# Autodesk Inventor assembly: mecanum_adaptive_trajectory
(part 2 of 2)
- 挿入:304 [Insert]: mecanum_encoder_plateD:1 ↔ mecanum_encoder_shaftD:1
- 挿入:305 [Insert]: mecanum_encoder_plateD:1 ↔ mecanum_encoder_shaftD:2
- 挿入:306 [Insert]: mecanum_encoder_plateD:1 ↔ mecanum_encoder_shaftD:3
- 挿入:307 [Insert]: mecanum_encoder_shaftD:1 ↔ mecanum_encoder_plateC:3
- 挿入:308 [Insert]: mecanum_encoder_shaftD:2 ↔ mecanum_encoder_plateC:3
- 挿入:309 [Insert]: mecanum_encoder_shaftD:3 ↔ mecanum_encoder_plateC:3
- メイト:77 [Mate]: mecanum_encoder_shaftA:1 ↔ mecanum_encoder_coupling:1
- メイト:78 [Mate] (4 mm): mecanum_encoder_plateC:1 ↔ mecanum_encoder_coupling:1
- メイト:79 [Mate]: Astuto_enc_wheel:2 ↔ mecanum_encoder_coupling:2
- メイト:80 [Mate] (5 mm): mecanum_encoder_plateC:2 ↔ mecanum_encoder_coupling:2
- メイト:81 [Mate]: Astuto_enc_wheel:2 ↔ mecanum_encoder_shaftE:1
- フラッシュ:6 [Flush] (10.609 mm): Astuto_enc_part3:2 ↔ Astuto_enc_part2:4
- フラッシュ:7 [Flush] (5 mm): mecanum_encoder_plateD:1 ↔ mecanum_encoder_shaftE:1
- [Insert]: E6A2-CW3C:3 ↔ mecanum_encoder_plateC:4
- [Insert]: E6A2-CW3C:3 ↔ mecanum_encoder_plateC:4
- [Mate]: Astuto_enc_part3:3 ↔ Astuto_enc_part2:7
- [Mate]: Astuto_enc_part3:4 ↔ Astuto_enc_part2:6
- [Mate] (0.2 mm): Astuto_enc_part3:3 ↔ Astuto_enc_part2:7
- [Mate] (0.2 mm): Astuto_enc_part3:4 ↔ Astuto_enc_part2:6
- [Insert]: Astuto_enc_part2:6 ↔ mecanum_encoder_plateD:2
- [Insert]: Astuto_enc_part2:7 ↔ mecanum_encoder_plateD:2
- [Insert]: Astuto_enc_part2:7 ↔ mecanum_encoder_plateD:2
- [Insert]: Astuto_enc_part2:6 ↔ mecanum_encoder_plateD:2
- [Mate]: Astuto_enc_wheel:3 ↔ mecanum_encoder_plateD:2
- [Insert]: mecanum_encoder_plateD:2 ↔ mecanum_encoder_shaftD:4
- [Insert]: mecanum_encoder_plateD:2 ↔ mecanum_encoder_shaftD:5
- [Insert]: mecanum_encoder_plateD:2 ↔ mecanum_encoder_shaftD:6
- [Insert]: mecanum_encoder_shaftD:4 ↔ mecanum_encoder_plateC:5
- [Insert]: mecanum_encoder_shaftD:5 ↔ mecanum_encoder_plateC:5
- [Insert]: mecanum_encoder_shaftD:6 ↔ mecanum_encoder_plateC:5
- [Mate]: Astuto_enc_wheel:3 ↔ mecanum_encoder_coupling:3
- [Mate] (5 mm): mecanum_encoder_plateC:4 ↔ mecanum_encoder_coupling:3
- [Mate]: Astuto_enc_wheel:3 ↔ mecanum_encoder_shaftE:2
- [Flush] (10.609 mm): Astuto_enc_part3:4 ↔ Astuto_enc_part2:6
- [Flush] (5 mm): mecanum_encoder_plateD:2 ↔ mecanum_encoder_shaftE:2
- 挿入:331 [Insert]: mecanum_flameD:1 ↔ Astuto_enc_part3:3
- 挿入:332 [Insert]: mecanum_flameD:2 ↔ Astuto_enc_part3:3
- 挿入:333 [Insert]: mecanum_flameD:2 ↔ Astuto_enc_part3:4
- 挿入:334 [Insert]: mecanum_flameD:1 ↔ Astuto_enc_part3:4
- メイト:91 [Mate] (5 mm): Astuto_enc_wheel:1 ↔ mecanum_encoder_plateA:1
- [Mate]: Astuto_enc_wheel:4 ↔ mecanum_encoder_shaftA:2
- [Mate]: mecanum_encoder_shaftA:2 ↔ mecanum_encoder_plateB:2
- [Mate]: Astuto_enc_part1:4 ↔ Astuto_enc_part2:8
- [Mate] (0.2 mm): Astuto_enc_part1:4 ↔ Astuto_enc_part2:8
- [Insert]: mecanum_encoder_plateB:2 ↔ Astuto_enc_part2:8
- [Insert]: mecanum_encoder_plateB:2 ↔ Astuto_enc_part2:8
- [Mate]: Astuto_enc_part1:5 ↔ Astuto_enc_part2:9
- [Insert]: mecanum_encoder_plateB:2 ↔ Astuto_enc_part2:9
- [Insert]: mecanum_encoder_plateB:2 ↔ Astuto_enc_part2:9
- [Mate] (0.2 mm): Astuto_enc_part1:5 ↔ Astuto_enc_part2:9
- [Flush] (17.307 mm): Astuto_enc_part1:4 ↔ Astuto_enc_part2:8
- [Mate]: mecanum_encoder_shaftA:2 ↔ mecanum_encoder_plateA:2
- [Insert]: mecanum_encoder_plateB:2 ↔ mecanum_encoder_shaftB:3
- [Insert]: mecanum_encoder_plateA:2 ↔ mecanum_encoder_shaftB:3
- [Insert]: mecanum_encoder_plateA:2 ↔ mecanum_encoder_shaftB:4
- [Insert]: E6A2-CW3C:4 ↔ mecanum_encoder_plateC:6
- [Insert]: E6A2-CW3C:4 ↔ mecanum_encoder_plateC:6
- [Mate]: mecanum_encoder_shaftA:2 ↔ E6A2-CW3C:4
- [Flush] (6 mm): mecanum_encoder_shaftA:2 ↔ mecanum_encoder_plateA:2
- [Insert]: mecanum_encoder_plateC:6 ↔ mecanum_encoder_shaftC:10
- [Insert]: mecanum_encoder_plateC:6 ↔ mecanum_encoder_shaftC:12
- [Insert]: mecanum_encoder_plateC:6 ↔ mecanum_encoder_shaftC:11
- [Mate]: mecanum_encoder_plateB:2 ↔ mecanum_encoder_shaftC:10
- [Insert]: mecanum_encoder_plateB:2 ↔ mecanum_encoder_shaftC:12
- [Insert]: mecanum_encoder_plateB:2 ↔ mecanum_encoder_shaftC:10
- [Insert]: mecanum_encoder_plateB:2 ↔ mecanum_encoder_shaftC:11
- [Mate]: mecanum_encoder_shaftA:2 ↔ mecanum_encoder_coupling:4
- [Mate] (4 mm): mecanum_encoder_plateC:6 ↔ mecanum_encoder_coupling:4
- [Mate] (5 mm): Astuto_enc_wheel:4 ↔ mecanum_encoder_plateA:2
- 挿入:350 [Insert]: mecanum_flameB_MIR:1 ↔ Astuto_enc_part1:4
- 挿入:351 [Insert]: mecanum_flameB_MIR:4 ↔ Astuto_enc_part1:4
- 挿入:352 [Insert]: mecanum_flameB_MIR:4 ↔ Astuto_enc_part1:5
- 挿入:353 [Insert]: mecanum_flameB_MIR:1 ↔ Astuto_enc_part1:5
- メイト:105 [Mate] (6.15 mm): Astuto_enc_wheel:2 ↔ mecanum_encoder_plateD:1
- メイト:106 [Mate] (6.15 mm): Astuto_enc_wheel:3 ↔ mecanum_encoder_plateD:2
- 挿入:354 [Insert]: mecanum_encoder_plateC:5 ↔ mecanum_encoder_shaftF:1
- 挿入:355 [Insert]: mecanum_encoder_plateC:4 ↔ mecanum_encoder_shaftF:1
- 挿入:356 [Insert]: mecanum_encoder_plateC:4 ↔ mecanum_encoder_shaftF:2
- 挿入:357 [Insert]: mecanum_encoder_plateC:4 ↔ mecanum_encoder_shaftF:3
- 挿入:358 [Insert]: mecanum_encoder_plateC:5 ↔ mecanum_encoder_shaftF:2
- 挿入:359 [Insert]: mecanum_encoder_plateC:5 ↔ mecanum_encoder_shaftF:3
- 挿入:360 [Insert]: mecanum_encoder_plateC:3 ↔ mecanum_encoder_shaftF:4
- 挿入:361 [Insert]: mecanum_encoder_plateC:2 ↔ mecanum_encoder_shaftF:4
- 挿入:362 [Insert]: mecanum_encoder_plateC:2 ↔ mecanum_encoder_shaftF:5
- 挿入:363 [Insert]: mecanum_encoder_plateC:2 ↔ mecanum_encoder_shaftF:6
- 挿入:364 [Insert]: mecanum_encoder_plateC:3 ↔ mecanum_encoder_shaftF:5
- 挿入:365 [Insert]: mecanum_encoder_plateC:3 ↔ mecanum_encoder_shaftF:6
- 挿入:372 [Insert]: mecanum_flameB_MIR:2 ↔ mecanum_flameF:1
- 挿入:373 [Insert]: mecanum_flameB_MIR:3 ↔ mecanum_flameF:1
- 挿入:374 [Insert]: mecanum_flameB_MIR:2 ↔ mecanum_flameF:2
- 挿入:375 [Insert]: mecanum_flameB_MIR:3 ↔ mecanum_flameF:2
- 挿入:377 [Insert]: mecanum_flameF:1 ↔ mecanum_LRF_flameA:1
- 挿入:379 [Insert]: mecanum_flameF:2 ↔ mecanum_LRF_flameA:2
- 挿入:384 [Insert]: LRF:1 ↔ mecanum_LRF_plate:1
- 挿入:385 [Insert]: LRF:1 ↔ mecanum_LRF_plate:1
- 挿入:386 [Insert]: LRF:1 ↔ mecanum_LRF_plate:1
- 挿入:387 [Insert]: LRF:1 ↔ mecanum_LRF_plate:1
- 挿入:388 [Insert]: mecanum_LRF_flameA:1 ↔ mecanum_LRF_plate:1
- 挿入:389 [Insert]: mecanum_LRF_flameA:1 ↔ mecanum_LRF_plate:1
- 挿入:390 [Insert]: mecanum_LRF_flameA:2 ↔ mecanum_LRF_plate:1
- 挿入:391 [Insert]: mecanum_LRF_flameA:2 ↔ mecanum_LRF_plate:1
- 挿入:392 [Insert]: mecanum_LRF_flameA:1 ↔ mecanum_gusset_plateA:1
- 挿入:393 [Insert]: mecanum_LRF_flameA:1 ↔ mecanum_gusset_plateA:1
- 挿入:394 [Insert]: mecanum_flameF:1 ↔ mecanum_LRF_flameB:1
- 挿入:395 [Insert]: mecanum_gusset_plateA:1 ↔ mecanum_LRF_flameB:1
- 挿入:396 [Insert]: mecanum_gusset_plateA:1 ↔ mecanum_LRF_flameB:1
- 挿入:397 [Insert]: mecanum_LRF_flameA:2 ↔ mecanum_gusset_plateA:2
- 挿入:398 [Insert]: mecanum_LRF_flameA:2 ↔ mecanum_gusset_plateA:2
- 挿入:399 [Insert]: mecanum_gusset_plateA:2 ↔ mecanum_LRF_flameB:2
- 挿入:400 [Insert]: mecanum_gusset_plateA:2 ↔ mecanum_LRF_flameB:2
- 挿入:401 [Insert]: mecanum_flameF:2 ↔ mecanum_LRF_flameB:2
- [Insert]: mecanum_flameF:3 ↔ mecanum_LRF_flameA:3
- [Insert]: mecanum_flameF:4 ↔ mecanum_LRF_flameA:4
- [Insert]: LRF:3 ↔ mecanum_LRF_plate:2
- [Insert]: LRF:3 ↔ mecanum_LRF_plate:2
- [Insert]: LRF:3 ↔ mecanum_LRF_plate:2
- [Insert]: LRF:3 ↔ mecanum_LRF_plate:2
- [Insert]: mecanum_LRF_flameA:3 ↔ mecanum_LRF_plate:2
- [Insert]: mecanum_LRF_flameA:3 ↔ mecanum_LRF_plate:2
- [Insert]: mecanum_LRF_flameA:4 ↔ mecanum_LRF_plate:2
- [Insert]: mecanum_LRF_flameA:4 ↔ mecanum_LRF_plate:2
- [Insert]: mecanum_LRF_flameA:3 ↔ mecanum_gusset_plateA:3
- [Insert]: mecanum_LRF_flameA:3 ↔ mecanum_gusset_plateA:3
- [Insert]: mecanum_flameF:3 ↔ mecanum_LRF_flameB:3
- [Insert]: mecanum_gusset_plateA:3 ↔ mecanum_LRF_flameB:3
- [Insert]: mecanum_gusset_plateA:3 ↔ mecanum_LRF_flameB:3
- [Insert]: mecanum_LRF_flameA:4 ↔ mecanum_gusset_plateA:4
- [Insert]: mecanum_LRF_flameA:4 ↔ mecanum_gusset_plateA:4
- [Insert]: mecanum_gusset_plateA:4 ↔ mecanum_LRF_flameB:4
- [Insert]: mecanum_gusset_plateA:4 ↔ mecanum_LRF_flameB:4
- [Insert]: mecanum_flameF:4 ↔ mecanum_LRF_flameB:4
- 挿入:422 [Insert]: mecanum_flameB:2 ↔ mecanum_flameF:3
- 挿入:423 [Insert]: mecanum_flameB:3 ↔ mecanum_flameF:3
- 挿入:424 [Insert]: mecanum_flameB:2 ↔ mecanum_flameF:4
- 挿入:425 [Insert]: mecanum_flameB:3 ↔ mecanum_flameF:4
- 挿入:426 [Insert]: mecanum_flameB_MIR:2 ↔ mecanum_LRF_flameA:2
- 挿入:427 [Insert]: mecanum_flameB_MIR:2 ↔ mecanum_LRF_flameA:1
- 挿入:428 [Insert]: mecanum_flameB:2 ↔ mecanum_LRF_flameA:3
- 挿入:429 [Insert]: mecanum_flameB:2 ↔ mecanum_LRF_flameA:4
- メイト:107 [Mate]: mecanum_angleA:2 ↔ mecanum_kusaA:2
- フラッシュ:13 [Flush]: mecanum_angleA:2 ↔ mecanum_kusaA:2
- フラッシュ:14 [Flush]: mecanum_angleA:2 ↔ mecanum_kusaA:2
- フラッシュ:15 [Flush]: mecanum_angleA:1 ↔ mecanum_kusaA:1
- フラッシュ:16 [Flush]: mecanum_angleA:1 ↔ mecanum_kusaA:1
- メイト:108 [Mate]: mecanum_angleA:1 ↔ mecanum_kusaA:1
- メイト:109 [Mate]: mecanum_angleB:2 ↔ mecanum_kusaB:1
- フラッシュ:17 [Flush]: mecanum_angleB:2 ↔ mecanum_kusaB:1
- フラッシュ:18 [Flush]: mecanum_angleB:2 ↔ mecanum_kusaB:1
- フラッシュ:19 [Flush]: mecanum_angleB:1 ↔ mecanum_kusaB:2
- フラッシュ:20 [Flush]: mecanum_angleB:1 ↔ mecanum_kusaB:2
- メイト:110 [Mate]: mecanum_angleB:1 ↔ mecanum_kusaB:2
- 挿入:430 [Insert]: mecanum_flameB:2 ↔ mecanum_flameG:1
- 挿入:431 [Insert]: mecanum_flameE:1 ↔ mecanum_flameG:1
- 挿入:432 [Insert]: motor_plate:1 ↔ mecanum_flameG:1
- 挿入:433 [Insert]: motor_plate:1 ↔ mecanum_flameG:1
- 挿入:434 [Insert]: mecanum_flameB:1 ↔ mecanum_flameG:1
- 挿入:435 [Insert]: mecanum_flameE:5 ↔ mecanum_flameG:1
- 挿入:436 [Insert]: mecanum_flameE_MIR:5 ↔ mecanum_flameG:1
- 挿入:437 [Insert]: mecanum_flameB_MIR:1 ↔ mecanum_flameG:1
- 挿入:438 [Insert]: motor_plate_MIR1:1 ↔ mecanum_flameG:1
- 挿入:439 [Insert]: motor_plate_MIR1:1 ↔ mecanum_flameG:1
- 挿入:440 [Insert]: mecanum_flameB_MIR:2 ↔ mecanum_flameG:1
- 挿入:441 [Insert]: mecanum_flameE_MIR:1 ↔ mecanum_flameG:1
- 挿入:442 [Insert]: mecanum_flameE:1 ↔ mecanum_flameG:2
- 挿入:443 [Insert]: mecanum_flameB:3 ↔ mecanum_flameG:2
- 挿入:444 [Insert]: motor_plate:1 ↔ mecanum_flameG:2
- 挿入:445 [Insert]: motor_plate:1 ↔ mecanum_flameG:2
- 挿入:446 [Insert]: mecanum_flameB:4 ↔ mecanum_flameG:2
- 挿入:447 [Insert]: mecanum_flameB:3 ↔ mecanum_flameG:2
- 挿入:448 [Insert]: mecanum_flameE:1 ↔ mecanum_flameG:2
- 挿入:449 [Insert]: mecanum_flameE:5 ↔ mecanum_flameG:2
- 挿入:450 [Insert]: mecanum_flameB_MIR:4 ↔ mecanum_flameG:2
- 挿入:451 [Insert]: mecanum_flameE_MIR:5 ↔ mecanum_flameG:2
- 挿入:452 [Insert]: motor_plate_MIR1:1 ↔ mecanum_flameG:2
- 挿入:453 [Insert]: motor_plate_MIR1:1 ↔ mecanum_flameG:2
- 挿入:454 [Insert]: mecanum_flameB_MIR:3 ↔ mecanum_flameG:2
- 挿入:455 [Insert]: mecanum_flameE_MIR:1 ↔ mecanum_flameG:2
- 挿入:456 [Insert]: mecanum_flameE_MIR:3 ↔ mecanum_flameG:3
- 挿入:457 [Insert]: mecanum_flameB_MIR:3 ↔ mecanum_flameG:3
- 挿入:458 [Insert]: motor_plate_MIR_MIR:1 ↔ mecanum_flameG:3
- 挿入:459 [Insert]: mecanum_flameE_MIR:6 ↔ mecanum_flameG:3
- 挿入:460 [Insert]: mecanum_flameB:4 ↔ mecanum_flameG:3
- 挿入:461 [Insert]: mecanum_flameE:6 ↔ mecanum_flameG:3
- 挿入:462 [Insert]: motor_plate_MIR:1 ↔ mecanum_flameG:3
- 挿入:463 [Insert]: motor_plate_MIR:1 ↔ mecanum_flameG:3
- 挿入:464 [Insert]: mecanum_flameB:3 ↔ mecanum_flameG:3
- 挿入:465 [Insert]: mecanum_flameB:3 ↔ mecanum_flameE:3
- 挿入:466 [Insert]: mecanum_flameE_MIR:3 ↔ mecanum_flameG:4
- 挿入:467 [Insert]: mecanum_flameB_MIR:2 ↔ mecanum_flameG:4
- 挿入:468 [Insert]: motor_plate_MIR_MIR:1 ↔ mecanum_flameG:4
- 挿入:469 [Insert]: motor_plate_MIR_MIR:1 ↔ mecanum_flameG:4
- 挿入:470 [Insert]: mecanum_flameB_MIR:1 ↔ mecanum_flameG:4
- 挿入:471 [Insert]: mecanum_flameE_MIR:6 ↔ mecanum_flameG:4
- 挿入:472 [Insert]: mecanum_flameB:1 ↔ mecanum_flameG:4
- 挿入:473 [Insert]: mecanum_flameE:6 ↔ mecanum_flameG:4
- 挿入:474 [Insert]: motor_plate_MIR:1 ↔ mecanum_flameG:4
- 挿入:475 [Insert]: motor_plate_MIR:1 ↔ mecanum_flameG:4
- 挿入:476 [Insert]: mecanum_flameB:2 ↔ mecanum_flameG:4
- 挿入:477 [Insert]: mecanum_flameE:3 ↔ mecanum_flameG:4
- 挿入:478 [Insert]: mecanum_flameG:4 ↔ mecanum_flameH:1
- 挿入:479 [Insert]: mecanum_flameG:1 ↔ mecanum_flameH:1
- 挿入:480 [Insert]: mecanum_flameG:4 ↔ mecanum_flameH:2
- 挿入:481 [Insert]: mecanum_flameG:1 ↔ mecanum_flameH:2
- 挿入:482 [Insert]: mecanum_flameH:1 ↔ mecanum_suction_motor_plate:1
- 挿入:483 [Insert]: mecanum_suction_motor_plate:1 ↔ mecanum_flameH:2
- 挿入:484 [Insert]: mecanum_flameH:1 ↔ mecanum_suction_motor_plate:1
- 挿入:485 [Insert]: mecanum_suction_motor_plate:1 ↔ mecanum_flameH:2
- 挿入:486 [Insert]: fan_冶具-01:1 ↔ mecanum_suction_motor_plate:1
- 挿入:487 [Insert]: fan_冶具-01:1 ↔ mecanum_suction_motor_plate:1
- 挿入:488 [Insert]: fan_冶具-01:1 ↔ mecanum_suction_motor_plate:1
- 挿入:489 [Insert]: fan_冶具-01:1 ↔ mecanum_suction_motor_plate:1
- 挿入:490 [Insert]: fan_冶具-01:1 ↔ mecanum_suction_motor_plate:1
- 挿入:491 [Insert]: fan_冶具-01:2 ↔ mecanum_suction_motor_plate:1
- 挿入:492 [Insert]: fan_冶具-01:2 ↔ mecanum_suction_motor_plate:1
- 挿入:493 [Insert]: fan_冶具-01:2 ↔ mecanum_suction_motor_plate:1
- 挿入:494 [Insert]: fan_冶具-01:2 ↔ mecanum_suction_motor_plate:1
- メイト:111 [Mate]: 14-KEY-RZ-735:1 ↔ mecanum_shaft:1
- メイト:112 [Mate]: 14-KEY-RZ-736_MIR:1 ↔ mecanum_shaft_MIR:1
- メイト:113 [Mate]: 14-KEY-RZ-736_MIR1:1 ↔ mecanum_shaft_MIR1:1
- メイト:114 [Mate]: 14-KEY-RZ-736_MIR_MIR:1 ↔ mecanum_shaft_MIR_MIR:1
## Named parameters: d291_d278 = 0 mm, d292_d280 = 0 mm, d293_d281 = 0 mm, d294_d282 = 0 mm, d295_d283 = 0 mm, d296_d288 = 0 mm, d297_d289 = 0 mm, d298_d290 = 0 mm, d306_d278 = 0 mm, d307_d280 = 0 mm, d308_d281 = 0 mm, d309_d282 = 0 mm, d310_d283 = 0 mm, d311_d288 = 0 mm, d312_d289 = 0 mm, d313_d290 = 0 mm, d314_d278 = 0 mm, d315_d280 = 0 mm, d316_d281 = 0 mm, d317_d282 = 0 mm, d318_d283 = 0 mm, d319_d288 = 0 mm, d320_d289 = 0 mm, d321_d290 = 0 mm, d343_d339 = 0 mm, d382_d368 = 0 mm, d383_d369 = 0 mm, d425_d423 = 10 mm, d426_d424 = 5 mm, d427_d402 = 0 mm, d428_d403 = 0 mm, d429_d404 = 0 mm, d430_d405 = 0 mm, d431_d406 = 0 mm, d432_d407 = 0 mm, d433_d397 = 0 mm, d434_d398 = 0 mm, d435_d399 = 0.2 mm, d436_d400 = 0.2 mm, d437_d401 = 0 mm, d438_d408 = 0 mm, d439_d409 = 0 mm, d440_d410 = 0 mm, d441_d411 = 0 mm, d447_d382_d368 = 0 mm, d448_d383_d369 = 0 mm, d450_d417 = 0 mm, d451_d418 = 5 mm, d452_d420 = 0 mm, d453_d421 = 10.609 mm, d454_d422 = 20 mm, d461_d415 = 0 mm, d462_d373 = 0 mm, d463_d374 = 0 mm, d464_d375 = 0 mm, d465_d376 = 0 mm, d466_d377 = 0 mm, d467_d378 = 0 mm, d468_d416 = 4 mm, d469_d460 = 5 mm, d470_d363 = 0 mm, d471_d365 = 0 mm, d472_d366 = 0 mm, d473_d367 = 0 mm, d474_d368 = 0 mm, d475_d369 = 0 mm, d476_d370 = 0 mm, d477_d371 = 6 mm, d478_d372 = 0 mm, d479_d336 = 0 mm, d480_d338 = 0 mm, d481_d339 = 0 mm, d482_d340 = 0.2 mm, d483_d341 = 0 mm, d484_d342 = 0 mm, d485_d343_d339 = 0 mm, d486_d345 = 0 mm, d487_d346 = 0 mm, d488_d358 = 0.2 mm, d489_d359 = 17.307 mm, d490_d360 = 15 mm, d491_d361 = 5 mm, d557_d542 = 0 mm, d558_d543 = 0 mm, d559_d544 = 0 mm, d560_d545 = 0 mm, d561_d546 = 0 mm, d562_d547 = 0 mm, d563_d548 = 0 mm, d564_d537 = 0 mm, d565_d539 = 0 mm, d566_d540 = 0 mm, d567_d541 = 0 mm, d568_d528 = 0 mm, d569_d530 = 0 mm, d570_d550 = 0 mm, d571_d551 = 0 mm, d572_d552 = 0 mm, d573_d553 = 0 mm, d574_d554 = 0 mm, d575_d555 = 0 mm, d576_d556 = 0 mm
